# Autodesk Inventor assembly: k1
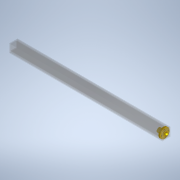
[picture p0: Inventor's stored thumbnail of the model, 180x180]
Saved by Autodesk Inventor 2020 (Build 240168000, 168)
## iProperties
Created: 2020-12-25
Part Number: k1
Document SubType Name: Assembly
Designer: Vikki
Author: Vikki
## Documents named in this file (4)
- D:\borewell rescuebot\pll manipulator files\sps manipulator\k1.iam
- D:\borewell rescuebot\pll manipulator files\sps manipulator\Part2.ipt
- D:\borewell rescuebot\pll manipulator files\sps manipulator\LeadScrew 8mm x 2mmPitch.ipt
- D:\borewell rescuebot\pll manipulator files\sps manipulator\LeadScrew Nut 8mm x 2mmPitch.ipt
## Components (3 placed, 3 different names)
1. Part2:1 — Mate:1
2. LeadScrew 8mm x 2mmPitch:1
3. LeadScrew Nut 8mm x 2mmPitch:1 — Mate:1
## Relationships (1: Mate 1)
- Mate:1: Part2:1 ↔ LeadScrew Nut 8mm x 2mmPitch:1
